# Autodesk Inventor assembly: Air puffs
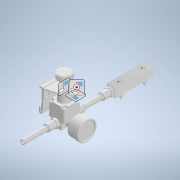
[picture p0: Inventor's stored thumbnail of the model, 180x180]
Saved by Autodesk Inventor 2021.2 (Build 252289000, 289)
## iProperties
Created: 2021-09-09
Part Number: Air puffs
Document SubType Name: Assembly
Designer: jl4459
Author: jl4459
## Documents named in this file (8)
- C:\Users\jl4459\Documents\Inventor\Training mini VR rig\Modules\Air puffs\Air puffs.iam
- C:\Users\jl4459\Documents\Inventor\Training mini VR rig\Modules\Air puffs\Parts\2227T21_Miniature Precision Compressed Air Regulator.ipt
- C:\Users\jl4459\Documents\Inventor\Training mini VR rig\Modules\Air puffs\Parts\2227T41_Mounting Bracket for Inline Mount 1 8 NPT Miniature Precision Compressed Air Regulator.ipt
- C:\Users\jl4459\Documents\Inventor\Training mini VR rig\Modules\Air puffs\Parts\2227T420_PRECISION NPT THREAD MINIATURE AIR REGULATOR.ipt
- C:\Users\jl4459\Documents\Inventor\Training mini VR rig\Modules\Air puffs\Parts\8961K106_MOUNTING ADAPTERS FOR DIN RAIL(1).ipt
- C:\Users\jl4459\Documents\Inventor\Training mini VR rig\Modules\Air puffs\Parts\5779K115_PUSH-TO-CONNECT TUBE FITTING FOR AIR.ipt
- C:\Users\jl4459\Documents\Inventor\Training mini VR rig\Modules\Air puffs\Control manifold.iam
- C:\Users\jl4459\Documents\Inventor\Training mini VR rig\Modules\Air puffs\Parts\5648K266_POLYURETHANE TUBING FOR WATER.ipt
## Components (9 placed, 7 different names)
1. 2227T21_Miniature Precision Compressed Air Regulator:1 — Mate:2, Mate:4, Insert:1, Insert:2, Insert:3
2. 2227T41_Mounting Bracket for Inline Mount 1 8 NPT Miniature Precision Compressed Air Regulator:2 — Mate:1, Mate:2, Mate:4, Flush:1, Flush:2
3. 2227T420_PRECISION NPT THREAD MINIATURE AIR REGULATOR:1 — Insert:3
4. 8961K106_MOUNTING ADAPTERS FOR DIN RAIL(1):1 — Mate:1, Flush:1, Flush:2
5. 5779K115_PUSH-TO-CONNECT TUBE FITTING FOR AIR:1 — Insert:1, Insert:5
6. 5779K115_PUSH-TO-CONNECT TUBE FITTING FOR AIR:2 — Insert:2, Insert:4
7. Control manifold:1 [sub-assembly] — Insert:6
8. 5648K266_POLYURETHANE TUBING FOR WATER:1 — Insert:5, Insert:6
9. 5648K266_POLYURETHANE TUBING FOR WATER:2 — Insert:4
## Relationships (11: Insert 6, Mate 3, Flush 2)
- Mate:1: 2227T41_Mounting Bracket for Inline Mount 1 8 NPT Miniature Precision Compressed Air Regulator:2 ↔ 8961K106_MOUNTING ADAPTERS FOR DIN RAIL(1):1
- Mate:2: 2227T21_Miniature Precision Compressed Air Regulator:1 ↔ 2227T41_Mounting Bracket for Inline Mount 1 8 NPT Miniature Precision Compressed Air Regulator:2
- Mate:4: 2227T21_Miniature Precision Compressed Air Regulator:1 ↔ 2227T41_Mounting Bracket for Inline Mount 1 8 NPT Miniature Precision Compressed Air Regulator:2
- Insert:1: 2227T21_Miniature Precision Compressed Air Regulator:1 ↔ 5779K115_PUSH-TO-CONNECT TUBE FITTING FOR AIR:1
- Insert:2: 2227T21_Miniature Precision Compressed Air Regulator:1 ↔ 5779K115_PUSH-TO-CONNECT TUBE FITTING FOR AIR:2
- Flush:1: 2227T41_Mounting Bracket for Inline Mount 1 8 NPT Miniature Precision Compressed Air Regulator:2 ↔ 8961K106_MOUNTING ADAPTERS FOR DIN RAIL(1):1
- Flush:2: 2227T41_Mounting Bracket for Inline Mount 1 8 NPT Miniature Precision Compressed Air Regulator:2 ↔ 8961K106_MOUNTING ADAPTERS FOR DIN RAIL(1):1
- Insert:3: 2227T21_Miniature Precision Compressed Air Regulator:1 ↔ 2227T420_PRECISION NPT THREAD MINIATURE AIR REGULATOR:1
- Insert:4 (-12.7 mm): 5779K115_PUSH-TO-CONNECT TUBE FITTING FOR AIR:2 ↔ 5648K266_POLYURETHANE TUBING FOR WATER:2
- Insert:5 (-12.7 mm): 5779K115_PUSH-TO-CONNECT TUBE FITTING FOR AIR:1 ↔ 5648K266_POLYURETHANE TUBING FOR WATER:1
- Insert:6 (-12.7 mm): Control manifold:1 ↔ 5648K266_POLYURETHANE TUBING FOR WATER:1
